# Autodesk Inventor assembly: KelleWelle1.ipt
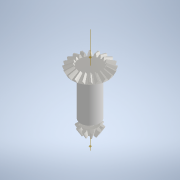
[picture p0: Inventor's stored thumbnail of the model, 180x180]
Saved by Autodesk Inventor 2021 (Build 250183000, 183)
## iProperties
Created: 2021-01-29
Part Number: KelleWelle1.ipt
Document SubType Name: Assembly
Designer: LETPJG
Author: LETPJG
## Documents named in this file (4)
- C:\Users\LETPJG\Documents\Vault\Gruppen\Gruppe 2\Entwurf\Amphibienfahrzeug\KelleWelle1.ipt.iam
- C:\Users\LETPJG\Documents\Vault\Gruppen\Gruppe 2\Entwurf\Amphibienfahrzeug\BauteilWelle2.ipt
- C:\Users\LETPJG\Documents\Vault\Gruppen\Gruppe 2\Entwurf\Amphibienfahrzeug\Planeten\Konstruktions-Assistent\Kegelrad12.ipt
- C:\Users\LETPJG\Documents\Vault\Gruppen\Gruppe 2\Entwurf\Amphibienfahrzeug\Planeten\Konstruktions-Assistent\Kegelrad22.ipt
## Components (3 placed, 3 different names)
1. BauteilWelle2:1 — Einfügen:1, Einfügen:2
2. Kegelrad1:1 — Einfügen:1
3. Kegelrad2:1 — Einfügen:2
## Relationships (2: Insert 2)
- Einfügen:1 [Insert]: BauteilWelle2:1 ↔ Kegelrad1:1
- Einfügen:2 [Insert]: BauteilWelle2:1 ↔ Kegelrad2:1
